# Autodesk Inventor assembly: Arm1.2ProtoAssembly
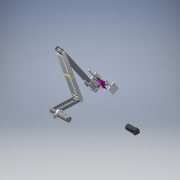
[picture p0: Inventor's stored thumbnail of the model, 180x180]
Saved by Autodesk Inventor 2017 (Build 210142000, 142)
## iProperties
Created: 2017-09-30
Part Number: Arm1.2ProtoAssembly
Document SubType Name: Assembly
Designer: User
Author: User
## Documents named in this file (11)
- C:\Robotics\CAD\2017-18_CAD\ArmProtoAssembly2.0.iam
- C:\Robotics\CAD\2017-18_CAD\ArmProto1.2.ipt
- C:\Robotics\CAD\COTSParts\Vex\REV-41-1097.iam
- C:\Robotics\CAD\COTSParts\Tetrix\39020_txm-servo mount horn.ipt
- C:\Robotics\CAD\2017-18_CAD\ArmProto2.2.ipt
- C:\Robotics\CAD\2017-18_CAD\ArmProto3.2.ipt
- C:\Robotics\CAD\COTSParts\Tetrix\tetrix-motor-mounts-1.snapshot.1\Tetrex 2pc motor mount.ipt
- C:\Robotics\CAD\COTSParts\Motors\Andymark 2964  NeveRest 40 Motor.ipt
- C:\Robotics\CAD\COTSParts\Fasteners\91259A533_ALLOY STEEL SHOULDER SCREW.ipt
- C:\Robotics\CAD\2017-18_CAD\Claw2017-18.iam
- C:\Robotics\CAD\COTSParts\Motors\REV-41-1300.ipt
## Components (13 placed, 10 different names)
1. ArmProto1.2:1 — Insert:2, Insert:10, Insert:11, Insert:13
2. REV-41-1097:1 [sub-assembly] — Insert:1, Insert:2, Insert:13
3. 39020_txm-servo mount horn:1 — Insert:1, Insert:8
4. ArmProto2.2:1 — Insert:7, Insert:8
5. ArmProto3.2:1 — Insert:5, Insert:12, Insert:14, Insert:15, Insert:16
6. REV-41-1097:2 [sub-assembly] — Insert:4, Insert:5, Insert:14
7. 39020_txm-servo mount horn:2 — Insert:4, Insert:7
8. Tetrex 2pc motor mount:1 — Insert:9
9. Andymark 2964  NeveRest 40 Motor:1 — Insert:9, Insert:11
10. 91259A533_ALLOY STEEL SHOULDER SCREW:1 — Insert:10
11. 91259A533_ALLOY STEEL SHOULDER SCREW:2 — Insert:12
12. Claw2017-18:1 [sub-assembly] — Insert:15, Insert:16
13. REV-41-1300:1
## Relationships (14: Insert 14)
- Insert:1: REV-41-1097:1 ↔ 39020_txm-servo mount horn:1
- Insert:2: ArmProto1.2:1 ↔ REV-41-1097:1
- Insert:4: REV-41-1097:2 ↔ 39020_txm-servo mount horn:2
- Insert:5: ArmProto3.2:1 ↔ REV-41-1097:2
- Insert:7: ArmProto2.2:1 ↔ 39020_txm-servo mount horn:2
- Insert:8: 39020_txm-servo mount horn:1 ↔ ArmProto2.2:1
- Insert:9: Tetrex 2pc motor mount:1 ↔ Andymark 2964  NeveRest 40 Motor:1
- Insert:10: ArmProto1.2:1 ↔ 91259A533_ALLOY STEEL SHOULDER SCREW:1
- Insert:11: ArmProto1.2:1 ↔ Andymark 2964  NeveRest 40 Motor:1
- Insert:12: ArmProto3.2:1 ↔ 91259A533_ALLOY STEEL SHOULDER SCREW:2
- Insert:13: ArmProto1.2:1 ↔ REV-41-1097:1
- Insert:14: ArmProto3.2:1 ↔ REV-41-1097:2
- Insert:15: ArmProto3.2:1 ↔ Claw2017-18:1
- Insert:16: ArmProto3.2:1 ↔ Claw2017-18:1
